# Autodesk Inventor assembly: stack
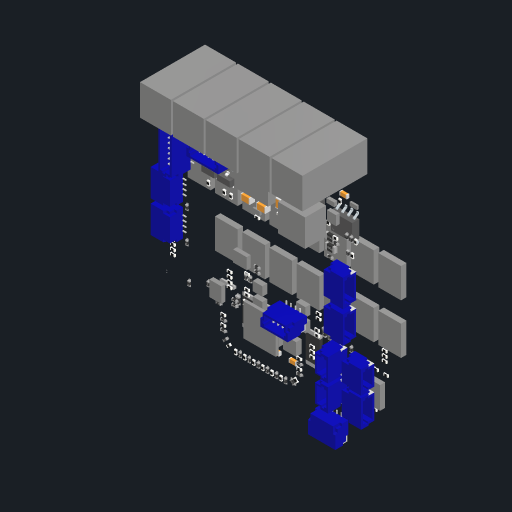
[picture p0: Inventor's stored thumbnail of the model, 512x512]
Saved by Autodesk Inventor 2023 (Build 270158000, 158)
## iProperties
Created: 2024-04-09
Part Number: stack
Document SubType Name: Assembly
Designer: szymo
Author: szymo
## Documents named in this file (3)
- C:\zRozne\roboilo\robots\wafel\3d_parts\stack.iam
- C:\zRozne\roboilo\robots\wafel\3d_parts\mcu.ipt
- C:\zRozne\roboilo\robots\wafel\3d_parts\Motor Driver.ipt
## Components (2 placed, 2 different names)
1. Motor Driver:1 — Mate:1, Flush:1, Flush:2
2. mcu:1 — Mate:1, Flush:1, Flush:2
## Relationships (3: Flush 2, Mate 1)
- Mate:1 (4 mm): Motor Driver:1 ↔ mcu:1
- Flush:1: Motor Driver:1 ↔ mcu:1
- Flush:2: Motor Driver:1 ↔ mcu:1
